# Autodesk Inventor assembly: handle
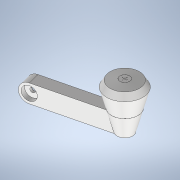
[picture p0: Inventor's stored thumbnail of the model, 180x180]
Saved by Autodesk Inventor 2021 (Build 250183000, 183)
## iProperties
Created: 2021-06-09
Part Number: handle
Document SubType Name: Assembly
Designer: teh18
Author: teh18
## iProperties of the stored document Rivet 005.ipt
Created: 2021-08-22
Part Number: Rivet 005
Material: Generic
Document SubType Name: Modeling
Designer: teh18
Density: 1 g/cm^3
Appearance: Default
Author: teh18
## iProperties of the stored document Rivet 002.ipt
Created: 2021-08-22
Part Number: Rivet 002
Material: Generic
Document SubType Name: Modeling
Designer: teh18
Density: 1 g/cm^3
Appearance: Default
Author: teh18
## iProperties of the stored document Rivet 006.ipt
Created: 2021-08-22
Part Number: Rivet 006
Material: Generic
Document SubType Name: Modeling
Designer: teh18
Density: 1 g/cm^3
Appearance: Default
Author: teh18
## iProperties of the stored document Seal 001.ipt
Created: 2021-08-22
Part Number: Seal 001
Material: Generic
Document SubType Name: Modeling
Designer: teh18
Density: 1 g/cm^3
Appearance: Default
Author: teh18
## iProperties of the stored document Ball 004.ipt
Created: 2021-08-22
Part Number: Ball 004
Material: Generic
Document SubType Name: Modeling
Designer: teh18
Density: 1 g/cm^3
Appearance: Default
Author: teh18
## iProperties of the stored document Outer Ring001.ipt
Created: 2021-08-22
Part Number: Outer Ring001
Material: Generic
Document SubType Name: Modeling
Designer: teh18
Density: 1 g/cm^3
Appearance: Default
Author: teh18
## iProperties of the stored document Ball 001.ipt
Created: 2021-08-22
Part Number: Ball 001
Material: Generic
Document SubType Name: Modeling
Designer: teh18
Density: 1 g/cm^3
Appearance: Default
Author: teh18
## iProperties of the stored document Inner Ring001.ipt
Created: 2021-08-22
Part Number: Inner Ring001
Material: Generic
Document SubType Name: Modeling
Designer: teh18
Density: 1 g/cm^3
Appearance: Default
Author: teh18
## iProperties of the stored document Cage 001.ipt
Created: 2021-08-22
Part Number: Cage 001
Material: Generic
Document SubType Name: Modeling
Designer: teh18
Density: 1 g/cm^3
Appearance: Default
Author: teh18
## iProperties of the stored document Ball 005.ipt
Created: 2021-08-22
Part Number: Ball 005
Material: Generic
Document SubType Name: Modeling
Designer: teh18
Density: 1 g/cm^3
Appearance: Default
Author: teh18
## iProperties of the stored document Ball 007.ipt
Created: 2021-08-22
Part Number: Ball 007
Material: Generic
Document SubType Name: Modeling
Designer: teh18
Density: 1 g/cm^3
Appearance: Default
Author: teh18
## iProperties of the stored document Cage 002.ipt
Created: 2021-08-22
Part Number: Cage 002
Material: Generic
Document SubType Name: Modeling
Designer: teh18
Density: 1 g/cm^3
Appearance: Default
Author: teh18
## iProperties of the stored document Ball 002.ipt
Created: 2021-08-22
Part Number: Ball 002
Material: Generic
Document SubType Name: Modeling
Designer: teh18
Density: 1 g/cm^3
Appearance: Default
Author: teh18
## iProperties of the stored document Rivet 007.ipt
Created: 2021-08-22
Part Number: Rivet 007
Material: Generic
Document SubType Name: Modeling
Designer: teh18
Density: 1 g/cm^3
Appearance: Default
Author: teh18
## iProperties of the stored document Rivet 003.ipt
Created: 2021-08-22
Part Number: Rivet 003
Material: Generic
Document SubType Name: Modeling
Designer: teh18
Density: 1 g/cm^3
Appearance: Default
Author: teh18
## iProperties of the stored document Seal 002.ipt
Created: 2021-08-22
Part Number: Seal 002
Material: Generic
Document SubType Name: Modeling
Designer: teh18
Density: 1 g/cm^3
Appearance: Default
Author: teh18
## iProperties of the stored document Ball 003.ipt
Created: 2021-08-22
Part Number: Ball 003
Material: Generic
Document SubType Name: Modeling
Designer: teh18
Density: 1 g/cm^3
Appearance: Default
Author: teh18
## iProperties of the stored document Ball 006.ipt
Created: 2021-08-22
Part Number: Ball 006
Material: Generic
Document SubType Name: Modeling
Designer: teh18
Density: 1 g/cm^3
Appearance: Default
Author: teh18
## iProperties of the stored document 608-2RS Skate Board Ball Bearing.iam
Created: 2021-08-02
Part Number: 608-2RS Skate Board Ball Bearing
Description: FreeCAD Model
Document SubType Name: Assembly
Designer: teh18
Authority: Unknown
Title: Open CASCADE Shape Model
Author: Author
Sending System: FreeCAD
Preprocessor: Open CASCADE STEP processor 7.5
## iProperties of the stored document Rivet 001.ipt
Created: 2021-08-22
Part Number: Rivet 001
Material: Generic
Document SubType Name: Modeling
Designer: teh18
Density: 1 g/cm^3
Appearance: Default
Author: teh18
## iProperties of the stored document Rivet 004.ipt
Created: 2021-08-22
Part Number: Rivet 004
Material: Generic
Document SubType Name: Modeling
Designer: teh18
Density: 1 g/cm^3
Appearance: Default
Author: teh18
## Documents named in this file (26)
- **C:\Users\teh18\OneDrive\BVE Controller\r68-bve-mascon\handle\handle.iam*LocalDocs*xAaaaqhbaAaaaaaaaAaaaq5utHc*Rivet 005.ipt
- **C:\Users\teh18\OneDrive\BVE Controller\r68-bve-mascon\handle\handle.iam*LocalDocs*xAaaaaibaAaaaaaaaAaaaqq2fYh*Rivet 002.ipt
- **C:\Users\teh18\OneDrive\BVE Controller\r68-bve-mascon\handle\handle.iam*LocalDocs*xAaaaa3aaAaaaaaaaAaaaqgqg2c*Rivet 006.ipt
- **C:\Users\teh18\OneDrive\BVE Controller\r68-bve-mascon\handle\handle.iam*LocalDocs*xAaaaa2caAaaaaaaaAaaaai4iEb*Seal 001.ipt
- **C:\Users\teh18\OneDrive\BVE Controller\r68-bve-mascon\handle\handle.iam*LocalDocs*xAaaaaabaAaaaaaaaAaaaauslBh*Ball 004.ipt
- **C:\Users\teh18\OneDrive\BVE Controller\r68-bve-mascon\handle\handle.iam*LocalDocs*xAaaaa4caAaaaaaaaAaaaqtjrMa*Outer Ring001.ipt
- **C:\Users\teh18\OneDrive\BVE Controller\r68-bve-mascon\handle\handle.iam*LocalDocs*xAaaaaeaaAaaaaaaaAaaaadpxMb*Ball 001.ipt
- **C:\Users\teh18\OneDrive\BVE Controller\r68-bve-mascon\handle\handle.iam*LocalDocs*xAaaaq2baAaaaaaaaAaaaa11mLh*Inner Ring001.ipt
- **C:\Users\teh18\OneDrive\BVE Controller\r68-bve-mascon\handle\handle.iam*LocalDocs*xAaaaamcaAaaaaaaaAaaaqy2fHd*Cage 001.ipt
- **C:\Users\teh18\OneDrive\BVE Controller\r68-bve-mascon\handle\handle.iam*LocalDocs*xAaaaaqbaAaaaaaaaAaaaqb1gIc*Ball 005.ipt
- **C:\Users\teh18\OneDrive\BVE Controller\r68-bve-mascon\handle\handle.iam*LocalDocs*xAaaaqeaaAaaaaaaaAaaaqayj0g*Ball 007.ipt
- **C:\Users\teh18\OneDrive\BVE Controller\r68-bve-mascon\handle\handle.iam*LocalDocs*xAaaaqddaAaaaaaaaAaaaqrvl2h*Cage 002.ipt
- **C:\Users\teh18\OneDrive\BVE Controller\r68-bve-mascon\handle\handle.iam*LocalDocs*xAaaaqddaAaaaaaaaAaaaq3n1Xg*Ball 002.ipt
- **C:\Users\teh18\OneDrive\BVE Controller\r68-bve-mascon\handle\handle.iam*LocalDocs*xAaaaqfaaAaaaaaaaAaaaa2osVh*Rivet 007.ipt
- **C:\Users\teh18\OneDrive\BVE Controller\r68-bve-mascon\handle\handle.iam*LocalDocs*xAaaaqybaAaaaaaaaAaaaax10Ra*Rivet 003.ipt
- **C:\Users\teh18\OneDrive\BVE Controller\r68-bve-mascon\handle\handle.iam*LocalDocs*xAaaaqvcaAaaaaaaaAaaaaxgrPa*Seal 002.ipt
- **C:\Users\teh18\OneDrive\BVE Controller\r68-bve-mascon\handle\handle.iam*LocalDocs*xAaaaqoaaAaaaaaaaAaaaqjzi4b*Ball 003.ipt
- **C:\Users\teh18\OneDrive\BVE Controller\r68-bve-mascon\handle\handle.iam*LocalDocs*xAaaaqkbaAaaaaaaaAaaaa022Th*Ball 006.ipt
- **C:\Users\teh18\OneDrive\BVE Controller\r68-bve-mascon\handle\handle.iam*LocalDocs*xAaaaqqdaAaaaaaaaAaaaqq1uAf*608-2RS Skate Board Ball Bearing.iam
- **C:\Users\teh18\OneDrive\BVE Controller\r68-bve-mascon\handle\handle.iam*LocalDocs*xAaaaqvdaAaaaaaaaAaaaazaoDd*Rivet 001.ipt
- **C:\Users\teh18\OneDrive\BVE Controller\r68-bve-mascon\handle\handle.iam*LocalDocs*xAaaaqzcaAaaaaaaaAaaaaizzOf*Rivet 004.ipt
- C:\Users\teh18\OneDrive\BVE Controller\r68-bve-mascon\handle\handle.iam
- C:\Users\teh18\OneDrive\BVE Controller\r68-bve-mascon\handle\metal.ipt
- C:\Users\teh18\OneDrive\BVE Controller\r68-bve-mascon\handle\free rotating sheath.ipt
- C:\Users\teh18\OneDrive\BVE Controller\r68-bve-mascon\handle\cap.ipt
- C:\Users\teh18\OneDrive\BVE Controller\608-skate-board-bearing-1.snapshot.14\608-2RS Skate Board Ball Bearing.step
## Components (4 placed, 4 different names)
1. metal:1 — Mate:1, Mate:2, Mate:3, Mate:4
2. cap:1 — Mate:1, Mate:2
3. free rotating sheath:2 — Mate:3, Mate:4, Mate:5, Mate:6
4. 608-2RS Skate Board Ball Bearing:1 [sub-assembly] — Mate:5, Mate:6
## Relationships (6: Mate 6)
- Mate:1: metal:1 ↔ cap:1
- Mate:2: metal:1 ↔ cap:1
- Mate:3: metal:1 ↔ free rotating sheath:2
- Mate:4: metal:1 ↔ free rotating sheath:2
- Mate:5: free rotating sheath:2 ↔ 608-2RS Skate Board Ball Bearing:1
- Mate:6: free rotating sheath:2 ↔ 608-2RS Skate Board Ball Bearing:1
